# Autodesk Inventor assembly: 61304021821 (rev1)
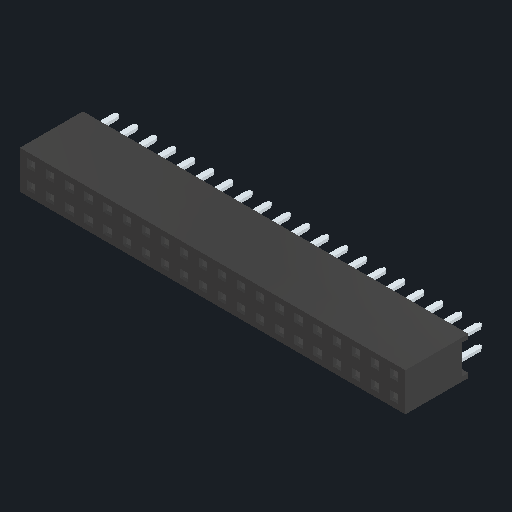
[picture p0: Inventor's stored thumbnail of the model, 512x512]
Saved by Autodesk Inventor 2022 (Build 260153000, 153)
## iProperties
Company: Unknown
Created: 2022-03-23
Part Number: 61304021821 (rev1)
Description: Unknown
Document SubType Name: Assembly
Designer: dvorakj
Sending System: Unknown
Preprocessor: PSStep 18.0.17
Title: C:/Users/quentin.payan/Documents/0-3D_2D/3D/Product Modification/613/6130xx21821/Construction_data/6130xx21821/61304021821/61304021821.stp
Author: Unknown
Revision Number: NONE
## Documents named in this file (3)
- C:\Users\dvorakj\Documents\Inventor\Bakalarka\Common\40\61304021821 (rev1).iam
- C:\Users\dvorakj\Documents\Inventor\Bakalarka\Common\40\6130xx21821_PIN.ipt
- C:\Users\dvorakj\Documents\Inventor\Bakalarka\Common\40\61304021821.ipt
## Components (41 placed, 41 different names)
1. NAUO1 — Flush:1
2. NAUO2
3. NAUO3 — Flush:1
4. NAUO4
5. NAUO5
6. NAUO6
7. NAUO7
8. NAUO8
9. NAUO9
10. NAUO10
11. NAUO11
12. NAUO12
13. NAUO13
14. NAUO14
15. NAUO15
16. NAUO16
17. NAUO17
18. NAUO18
19. NAUO19
20. NAUO20
21. NAUO21
22. NAUO22
23. NAUO23
24. NAUO24
25. NAUO25
26. NAUO26
27. NAUO27
28. NAUO28
29. NAUO29
30. NAUO30
31. NAUO31
32. NAUO32
33. NAUO33
34. NAUO34
35. NAUO35
36. NAUO36
37. NAUO37
38. NAUO38
39. NAUO39
40. NAUO40
41. NAUO41
## Relationships (1: Flush 1)
- Flush:1: NAUO1 ↔ NAUO3
